# Autodesk Inventor assembly: Mellie Cart V2
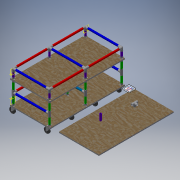
[picture p0: Inventor's stored thumbnail of the model, 180x180]
Saved by Autodesk Inventor 2018.2 (Build 222227000, 227)
## iProperties
Created: 2018-02-05
Part Number: Mellie Cart V2
Document SubType Name: Assembly
Designer: owner
Author: owner
## Documents named in this file (15)
- Z:\The Pickle\Final Carts\Mellie Cart\Mellie Cart V2.iam
- Z:\The Pickle\Final Carts\Mellie Cart\Plywood Base - Bottom.ipt
- Z:\The Pickle\Inventor Pipe Parts\Formufit Fittings\Wood Mount 1 Inch.ipt
- Z:\The Pickle\Inventor Pipe Parts\Formufit Fittings\Tee 1 Inch.ipt
- Z:\The Pickle\Inventor Pipe Parts\Formufit Fittings\4-way Tee 1 Inch.ipt
- Z:\The Pickle\Inventor Pipe Parts\Formufit Fittings\5-way 1 Inch.ipt
- Z:\The Pickle\Inventor Pipe Parts\Formufit Fittings\Cross 1 Inch.ipt
- Z:\The Pickle\Inventor Pipe Parts\Formufit Fittings\3-way 90 1 Inch.ipt
- Z:\The Pickle\Final Carts\Mellie Cart\Pipe 1.ipt
- Z:\The Pickle\Final Carts\Mellie Cart\Pipe 2.ipt
- Z:\The Pickle\Final Carts\Mellie Cart\Pipe 3.ipt
- Z:\The Pickle\Final Carts\Mellie Cart\Pipe 4.ipt
- Z:\The Pickle\Final Carts\Mellie Cart\Pipe 5.ipt
- Z:\The Pickle\Final Carts\Eye Bolt and Nut.iam
- Z:\The Pickle\Final Carts\WHEELS.ipt
## Components (83 placed, 14 different names)
1. Plywood Base - Bottom:1 — Mate:1, Tangent:1, Tangent:2, Flush:7, Flush:8, Mate:17, Tangent:5, Tangent:6, Flush:47, Flush:48, Flush:49, Mate:21
2. Wood Mount 1 Inch:1 — Mate:1, Tangent:1, Tangent:2, Insert:1, Flush:6
3. Wood Mount 1 Inch:2 — Insert:7, Flush:5
4. Wood Mount 1 Inch:3 — Insert:29, Flush:4
5. Wood Mount 1 Inch:4 — Insert:30, Flush:3
6. Wood Mount 1 Inch:5 — Insert:31, Flush:2
7. Wood Mount 1 Inch:6 — Insert:32, Flush:1, Tangent:6
8. Wood Mount 1 Inch:7 — Insert:33, Mate:17, Tangent:5
9. Wood Mount 1 Inch:8 — Insert:34, Flush:5
10. Wood Mount 1 Inch:9 — Insert:35, Flush:4
11. Wood Mount 1 Inch:10 — Insert:36, Flush:6, Mate:2
12. Wood Mount 1 Inch:11 — Insert:37, Flush:3
13. Wood Mount 1 Inch:12 — Insert:38, Flush:2
14. Wood Mount 1 Inch:13 — Insert:39, Flush:1
15. Wood Mount 1 Inch:14 — Insert:40
16. Wood Mount 1 Inch:15 — Mate:3, Tangent:3, Tangent:4, Insert:41
17. Wood Mount 1 Inch:16 — Insert:56
18. Wood Mount 1 Inch:17 — Insert:57
19. Wood Mount 1 Inch:19 — Insert:59
20. Wood Mount 1 Inch:21 — Insert:61
21. Wood Mount 1 Inch:25 — Insert:65
22. Tee 1 Inch:1 — Insert:23, Insert:24, Insert:25
23. Tee 1 Inch:3 — Insert:14, Insert:15, Insert:17
24. Tee 1 Inch:4 — Insert:2, Insert:3, Insert:4, Flush:22
25. 4-way Tee 1 Inch:1 — Insert:21, Insert:22, Insert:26, Insert:27
26. 4-way Tee 1 Inch:2 — Insert:106, Insert:107, Insert:109, Insert:110
27. 4-way Tee 1 Inch:3 — Insert:5, Insert:6, Insert:8, Insert:28
28. 5-way 1 Inch:1 — Insert:9, Insert:10, Insert:11, Insert:19, Insert:20
29. Cross 1 Inch:1 — Insert:12, Insert:13, Insert:16, Insert:18
30. 3-way 90 1 Inch:1 — Insert:48, Insert:49, Insert:76
31. 3-way 90 1 Inch:4 — Insert:50, Insert:51, Insert:77
32. 3-way 90 1 Inch:5 — Insert:85, Insert:99, Insert:108, Flush:24
33. 3-way 90 1 Inch:6 — Insert:87, Insert:100, Insert:101
34. Pipe 1:1 — Insert:22, Insert:23
35. Pipe 1:2 — Insert:4, Insert:5
36. Pipe 1:5 — Insert:49, Insert:50
37. Pipe 2:1 — Insert:28, Insert:34
38. Pipe 2:2 — Insert:26, Insert:32
39. Pipe 2:3 — Insert:18, Insert:37
40. Pipe 2:4 — Insert:16, Insert:30
41. Pipe 2:5 — Insert:15, Insert:31
42. Pipe 2:6 — Insert:25, Insert:40
43. Pipe 2:7 — Insert:24, Insert:33
44. Pipe 2:8 — Insert:10, Insert:29
45. Pipe 2:9 — Insert:17, Insert:38
46. Pipe 2:10 — Insert:3, Insert:36
47. Pipe 2:11 — Insert:6, Insert:7
48. Pipe 2:12 — Insert:19, Insert:35
49. Pipe 2:13 — Insert:1, Insert:2
50. Pipe 2:14 — Insert:27, Insert:39
51. Pipe 3:1 — Insert:11, Insert:12
52. Pipe 3:2 — Insert:13, Insert:14
53. Pipe 4:1 — Insert:8, Insert:9
54. Pipe 4:4 — Insert:51, Insert:110
55. Pipe 4:5 — Insert:101, Insert:103
56. Pipe 4:6 — Insert:48, Insert:104
57. Pipe 4:7 — Insert:20, Insert:21
58. Pipe 5:1 — Insert:65, Insert:77
59. Pipe 5:4 — Insert:61, Insert:76
60. Pipe 5:6 — Insert:59, Insert:107
61. Pipe 5:7 — Insert:41, Insert:99
62. Pipe 5:8 — Insert:56, Insert:100
63. Pipe 5:9 — Insert:57, Insert:102
64. Plywood Base - Bottom:2 — Mate:2, Flush:7, Flush:8, Mate:3, Tangent:3, Tangent:4
65. Pipe 1:6 — Insert:85, Insert:87
66. 4-way Tee 1 Inch:4 — Insert:102, Insert:103, Insert:104, Insert:105
67. Pipe 1:7 — Insert:105, Insert:106
68. Pipe 4:8 — Insert:108, Insert:109
69. Eye Bolt and Nut:1 [sub-assembly] — Flush:22, Flush:25, Flush:26, Mate:15, Flush:27
70. Eye Bolt and Nut:4 [sub-assembly] — Flush:24, Flush:25, Flush:26, Flush:28
71. Eye Bolt and Nut:5 [sub-assembly] — Mate:15, Flush:27, Mate:16, Flush:29
72. Eye Bolt and Nut:8 [sub-assembly] — Flush:28, Mate:16, Flush:29
73. WHEELS:1 — Flush:30, Flush:35, Flush:37, Flush:40, Flush:49, Mate:21
74. WHEELS:2 — Flush:30, Flush:34, Flush:37, Mate:18, Flush:47, Flush:48
75. WHEELS:3 — Flush:31, Flush:34, Flush:36, Flush:46, Mate:18, Mate:20
76. WHEELS:4 — Flush:32, Flush:38, Flush:45, Flush:46, Mate:19, Mate:20
77. WHEELS:5 — Flush:33, Flush:44, Flush:45, Mate:19
78. WHEELS:6 — Flush:33, Flush:42, Flush:43, Flush:44
79. WHEELS:7 — Flush:32, Flush:38, Flush:39, Flush:41, Flush:42, Flush:43
80. WHEELS:8 — Flush:31, Flush:35, Flush:36, Flush:39, Flush:40, Flush:41
81. 4-way Tee 1 Inch:5
82. Pipe 5:10
83. Plywood Base - Bottom:3
## Relationships (117: Insert 66, Flush 35, Mate 10, Tangent 6)
- Mate:1: Plywood Base - Bottom:1 ↔ Wood Mount 1 Inch:1
- Tangent:1: Plywood Base - Bottom:1 ↔ Wood Mount 1 Inch:1
- Tangent:2: Plywood Base - Bottom:1 ↔ Wood Mount 1 Inch:1
- Insert:1: Wood Mount 1 Inch:1 ↔ Pipe 2:13
- Insert:2: Tee 1 Inch:4 ↔ Pipe 2:13
- Insert:3: Tee 1 Inch:4 ↔ Pipe 2:10
- Insert:4: Tee 1 Inch:4 ↔ Pipe 1:2
- Insert:5: 4-way Tee 1 Inch:3 ↔ Pipe 1:2
- Insert:6: 4-way Tee 1 Inch:3 ↔ Pipe 2:11
- Insert:7: Wood Mount 1 Inch:2 ↔ Pipe 2:11
- Insert:8: 4-way Tee 1 Inch:3 ↔ Pipe 4:1
- Insert:9: 5-way 1 Inch:1 ↔ Pipe 4:1
- Insert:10: 5-way 1 Inch:1 ↔ Pipe 2:8
- Insert:11: 5-way 1 Inch:1 ↔ Pipe 3:1
- Insert:12: Cross 1 Inch:1 ↔ Pipe 3:1
- Insert:13: Cross 1 Inch:1 ↔ Pipe 3:2
- Insert:14: Tee 1 Inch:3 ↔ Pipe 3:2
- Insert:15: Tee 1 Inch:3 ↔ Pipe 2:5
- Insert:16: Cross 1 Inch:1 ↔ Pipe 2:4
- Insert:17: Tee 1 Inch:3 ↔ Pipe 2:9
- Insert:18: Cross 1 Inch:1 ↔ Pipe 2:3
- Insert:19: 5-way 1 Inch:1 ↔ Pipe 2:12
- Insert:20: 5-way 1 Inch:1 ↔ Pipe 4:7
- Insert:21: 4-way Tee 1 Inch:1 ↔ Pipe 4:7
- Insert:22: 4-way Tee 1 Inch:1 ↔ Pipe 1:1
- Insert:23: Tee 1 Inch:1 ↔ Pipe 1:1
- Insert:24: Tee 1 Inch:1 ↔ Pipe 2:7
- Insert:25: Tee 1 Inch:1 ↔ Pipe 2:6
- Insert:26: 4-way Tee 1 Inch:1 ↔ Pipe 2:2
- Insert:27: 4-way Tee 1 Inch:1 ↔ Pipe 2:14
- Insert:28: 4-way Tee 1 Inch:3 ↔ Pipe 2:1
- Insert:29: Wood Mount 1 Inch:3 ↔ Pipe 2:8
- Insert:30: Wood Mount 1 Inch:4 ↔ Pipe 2:4
- Insert:31: Wood Mount 1 Inch:5 ↔ Pipe 2:5
- Insert:32: Wood Mount 1 Inch:6 ↔ Pipe 2:2
- Insert:33: Wood Mount 1 Inch:7 ↔ Pipe 2:7
- Insert:34: Wood Mount 1 Inch:8 ↔ Pipe 2:1
- Insert:35: Wood Mount 1 Inch:9 ↔ Pipe 2:12
- Insert:36: Wood Mount 1 Inch:10 ↔ Pipe 2:10
- Insert:37: Wood Mount 1 Inch:11 ↔ Pipe 2:3
- Insert:38: Wood Mount 1 Inch:12 ↔ Pipe 2:9
- Insert:39: Wood Mount 1 Inch:13 ↔ Pipe 2:14
- Insert:40: Wood Mount 1 Inch:14 ↔ Pipe 2:6
- Flush:1: Wood Mount 1 Inch:6 ↔ Wood Mount 1 Inch:13
- Flush:2: Wood Mount 1 Inch:5 ↔ Wood Mount 1 Inch:12
- Flush:3: Wood Mount 1 Inch:4 ↔ Wood Mount 1 Inch:11
- Flush:4: Wood Mount 1 Inch:3 ↔ Wood Mount 1 Inch:9
- Flush:5: Wood Mount 1 Inch:2 ↔ Wood Mount 1 Inch:8
- Flush:6: Wood Mount 1 Inch:1 ↔ Wood Mount 1 Inch:10
- Mate:2: Wood Mount 1 Inch:10 ↔ Plywood Base - Bottom:2
- Flush:7: Plywood Base - Bottom:1 ↔ Plywood Base - Bottom:2
- Flush:8: Plywood Base - Bottom:1 ↔ Plywood Base - Bottom:2
- Mate:3: Wood Mount 1 Inch:15 ↔ Plywood Base - Bottom:2
- Tangent:3: Wood Mount 1 Inch:15 ↔ Plywood Base - Bottom:2
- Tangent:4: Wood Mount 1 Inch:15 ↔ Plywood Base - Bottom:2
- Insert:41: Wood Mount 1 Inch:15 ↔ Pipe 5:7
- Insert:48: 3-way 90 1 Inch:1 ↔ Pipe 4:6
- Insert:49: 3-way 90 1 Inch:1 ↔ Pipe 1:5
- Insert:50: 3-way 90 1 Inch:4 ↔ Pipe 1:5
- Insert:51: 3-way 90 1 Inch:4 ↔ Pipe 4:4
- Insert:56: Wood Mount 1 Inch:16 ↔ Pipe 5:8
- Insert:57: Wood Mount 1 Inch:17 ↔ Pipe 5:9
- Insert:59: Wood Mount 1 Inch:19 ↔ Pipe 5:6
- Insert:61: Wood Mount 1 Inch:21 ↔ Pipe 5:4
- Insert:65: Wood Mount 1 Inch:25 ↔ Pipe 5:1
- Insert:76: 3-way 90 1 Inch:1 ↔ Pipe 5:4
- Insert:77: 3-way 90 1 Inch:4 ↔ Pipe 5:1
- Insert:85: 3-way 90 1 Inch:5 ↔ Pipe 1:6
- Insert:87: 3-way 90 1 Inch:6 ↔ Pipe 1:6
- Insert:99: 3-way 90 1 Inch:5 ↔ Pipe 5:7
- Insert:100: 3-way 90 1 Inch:6 ↔ Pipe 5:8
- Insert:101: 3-way 90 1 Inch:6 ↔ Pipe 4:5
- Insert:102: Pipe 5:9 ↔ 4-way Tee 1 Inch:4
- Insert:103: Pipe 4:5 ↔ 4-way Tee 1 Inch:4
- Insert:104: Pipe 4:6 ↔ 4-way Tee 1 Inch:4
- Insert:105: 4-way Tee 1 Inch:4 ↔ Pipe 1:7
- Insert:106: 4-way Tee 1 Inch:2 ↔ Pipe 1:7
- Insert:107: 4-way Tee 1 Inch:2 ↔ Pipe 5:6
- Insert:108: 3-way 90 1 Inch:5 ↔ Pipe 4:8
- Insert:109: 4-way Tee 1 Inch:2 ↔ Pipe 4:8
- Insert:110: 4-way Tee 1 Inch:2 ↔ Pipe 4:4
- Flush:22 (-25.4 mm): Tee 1 Inch:4 ↔ Eye Bolt and Nut:1
- Flush:24 (-25.4 mm): 3-way 90 1 Inch:5 ↔ Eye Bolt and Nut:4
- Flush:25: Eye Bolt and Nut:1 ↔ Eye Bolt and Nut:4
- Flush:26: Eye Bolt and Nut:1 ↔ Eye Bolt and Nut:4
- Mate:15: Eye Bolt and Nut:1 ↔ Eye Bolt and Nut:5
- Flush:27: Eye Bolt and Nut:1 ↔ Eye Bolt and Nut:5
- Flush:28: Eye Bolt and Nut:4 ↔ Eye Bolt and Nut:8
- Mate:16: Eye Bolt and Nut:5 ↔ Eye Bolt and Nut:8
- Flush:29: Eye Bolt and Nut:5 ↔ Eye Bolt and Nut:8
- Flush:30: WHEELS:1 ↔ WHEELS:2
- Flush:31: WHEELS:3 ↔ WHEELS:8
- Flush:32: WHEELS:4 ↔ WHEELS:7
- Flush:33: WHEELS:5 ↔ WHEELS:6
- Flush:34: WHEELS:2 ↔ WHEELS:3
- Flush:35: WHEELS:1 ↔ WHEELS:8
- Flush:36: WHEELS:3 ↔ WHEELS:8
- Flush:37: WHEELS:1 ↔ WHEELS:2
- Flush:38: WHEELS:4 ↔ WHEELS:7
- Flush:39: WHEELS:7 ↔ WHEELS:8
- Flush:40: WHEELS:1 ↔ WHEELS:8
- Flush:41: WHEELS:7 ↔ WHEELS:8
- Flush:42: WHEELS:6 ↔ WHEELS:7
- Flush:43: WHEELS:6 ↔ WHEELS:7
- Flush:44: WHEELS:5 ↔ WHEELS:6
- Flush:45: WHEELS:4 ↔ WHEELS:5
- Flush:46: WHEELS:3 ↔ WHEELS:4
- Mate:17: Plywood Base - Bottom:1 ↔ Wood Mount 1 Inch:7
- Tangent:5: Plywood Base - Bottom:1 ↔ Wood Mount 1 Inch:7
- Tangent:6: Plywood Base - Bottom:1 ↔ Wood Mount 1 Inch:6
- Mate:18 (363.2031 mm): WHEELS:2 ↔ WHEELS:3
- Mate:19 (363.2031 mm): WHEELS:4 ↔ WHEELS:5
- Mate:20 (363.2031 mm): WHEELS:3 ↔ WHEELS:4
- Flush:47: Plywood Base - Bottom:1 ↔ WHEELS:2
- Flush:48: Plywood Base - Bottom:1 ↔ WHEELS:2
- Flush:49: Plywood Base - Bottom:1 ↔ WHEELS:1
- Mate:21: Plywood Base - Bottom:1 ↔ WHEELS:1
